# Autodesk Inventor assembly: Drive Roller Assembly 3 (Lexan)
(part 2 of 2)
- Flush:42: Hex Shaft Collar 3-8 in (7552K300):3 ↔ Hex Shaft 3-8 in (am-0855):4
- Mate:1246: Vex Pro 1x1 rectangular tubing 14 in length:5 ↔ Vex Pro T gusset - OUT OF STOCK 1192014:3
- Mate:1247: Vex Pro 1x1 rectangular tubing 14 in length:5 ↔ Vex Pro T gusset - OUT OF STOCK 1192014:3
- Mate:1248: Vex Pro 1x1 rectangular tubing 14 in length:5 ↔ Vex Pro T gusset - OUT OF STOCK 1192014:3
- Mate:1249: Vex Pro 1x1 rectangular tubing 4 in length:1 ↔ Vex Pro T gusset - OUT OF STOCK 1192014:3
- Mate:1250: Vex Pro 1x1 rectangular tubing 14 in length:5 ↔ Vex Pro T gusset - OUT OF STOCK 1192014:4
- Mate:1251: Vex Pro 1x1 rectangular tubing 14 in length:5 ↔ Vex Pro T gusset - OUT OF STOCK 1192014:4
- Mate:1252: Vex Pro 1x1 rectangular tubing 14 in length:5 ↔ Vex Pro T gusset - OUT OF STOCK 1192014:4
- Mate:1253: Vex Pro 1x1 rectangular tubing 4 in length:1 ↔ Vex Pro T gusset - OUT OF STOCK 1192014:4
- Mate:1254: Vex Pro 1x1 rectangular tubing 14 in length:6 ↔ Vex Pro T gusset - OUT OF STOCK 1192014:5
- Mate:1255: Vex Pro 1x1 rectangular tubing 14 in length:6 ↔ Vex Pro T gusset - OUT OF STOCK 1192014:5
- Mate:1256: Vex Pro 1x1 rectangular tubing 14 in length:6 ↔ Vex Pro T gusset - OUT OF STOCK 1192014:5
- Mate:1257: Vex Pro 1x1 rectangular tubing 4 in length:2 ↔ Vex Pro T gusset - OUT OF STOCK 1192014:5
- Mate:1258: Vex Pro 1x1 rectangular tubing 4 in length:1 ↔ Vex Pro T gusset - OUT OF STOCK 1192014:3
- Mate:1259: Vex Pro 1x1 rectangular tubing 4 in length:2 ↔ Vex Pro T gusset - OUT OF STOCK 1192014:5
- Mate:1260: Vex Pro 1x1 rectangular tubing 14 in length:6 ↔ Vex Pro T gusset - OUT OF STOCK 1192014:6
- Mate:1261: Vex Pro 1x1 rectangular tubing 14 in length:6 ↔ Vex Pro T gusset - OUT OF STOCK 1192014:6
- Mate:1262: Vex Pro 1x1 rectangular tubing 14 in length:6 ↔ Vex Pro T gusset - OUT OF STOCK 1192014:6
- Mate:1263: Vex Pro 1x1 rectangular tubing 4 in length:2 ↔ Vex Pro T gusset - OUT OF STOCK 1192014:6
- Mate:1264: Vex Pro 1x1 rectangular tubing 4 in length:2 ↔ Vex Pro T gusset - OUT OF STOCK 1192014:6
- Mate:1265: Vex Pro 1x1 rectangular tubing 4 in length:1 ↔ Vex Pro T gusset - OUT OF STOCK 1192014:3
- Mate:1266: Hex Spacer:3 ↔ Clamp with Piston Assembly (new):1
- Mate:1267: Vex Pro 1x1 rectangular tubing 21.375 in length:1 ↔ Roller Crossbar Gusset (Custom):5
- Mate:1268: Vex Pro 1x1 rectangular tubing 21.375 in length:1 ↔ Roller Crossbar Gusset (Custom):5
- Mate:1269: Vex Pro 1x1 rectangular tubing 21.375 in length:1 ↔ Roller Crossbar Gusset (Custom):5
- Mate:1272: Vex Pro 1x1 rectangular tubing 14 in length:5 ↔ Roller Piston 4 Mount:1
- Mate:1273: Vex Pro 1x1 rectangular tubing 14 in length:5 ↔ Roller Piston 4 Mount:1
- Mate:1274: Vex Pro 1x1 rectangular tubing 14 in length:5 ↔ Roller Piston 4 Mount:1
- Mate:1275: Vex Pro 1x1 rectangular tubing 14 in length:6 ↔ Roller Piston 4 Mount:2
- Mate:1276: Vex Pro 1x1 rectangular tubing 14 in length:6 ↔ Roller Piston 4 Mount:2
- Mate:1277: Vex Pro 1x1 rectangular tubing 14 in length:6 ↔ Roller Piston 4 Mount:2
- Mate:1278: Roller Piston 4 Mount:2 ↔ Roller Piston 4 (.5 and 1 in Stroke, 9-16 in Bore):1
- Mate:1279: Roller Piston 4 Mount:2 ↔ Roller Piston 4 (.5 and 1 in Stroke, 9-16 in Bore):1
- Mate:1280: Roller Piston 4 Mount:1 ↔ Roller Piston 4 (.5 and 1 in Stroke, 9-16 in Bore):2
- Mate:1281: Roller Piston 4 Mount:1 ↔ Roller Piston 4 (.5 and 1 in Stroke, 9-16 in Bore):2
- Mate:1282: Bracket:3 ↔ Roller Piston 4 (.5 and 1 in Stroke, 9-16 in Bore):2
- Mate:1283: Shaft Collar 3-16 in ID (6435K510):2 ↔ Roller Piston 4 (.5 and 1 in Stroke, 9-16 in Bore):2
- Mate:1284: Shaft Collar 3-16 in ID (6435K510):1 ↔ Roller Piston 4 (.5 and 1 in Stroke, 9-16 in Bore):2
- Mate:1285: Bracket:4 ↔ Roller Piston 4 (.5 and 1 in Stroke, 9-16 in Bore):1
- Mate:1286: Shaft Collar 3-16 in ID (6435K510):4 ↔ Roller Piston 4 (.5 and 1 in Stroke, 9-16 in Bore):1
- Mate:1287: Shaft Collar 3-16 in ID (6435K510):3 ↔ Roller Piston 4 (.5 and 1 in Stroke, 9-16 in Bore):1
- Mate:1292: Vex Pro 1x1 rectangular tubing 14 in length:6 ↔ Vex Pro T gusset - OUT OF STOCK 1192014:8
- Mate:1293: Vex Pro 1x1 rectangular tubing 14 in length:6 ↔ Vex Pro T gusset - OUT OF STOCK 1192014:8
- Mate:1294: Vex Pro 1x1 rectangular tubing 14 in length:6 ↔ Vex Pro T gusset - OUT OF STOCK 1192014:8
- Mate:1300: Hex Shaft Collar 1-2 in (7552K500):19 ↔ Hex Shaft 1-2 in 5 in long (am-0856):1
- Mate:1301: Hex Shaft Collar 1-2 in (7552K500):18 ↔ Hex Shaft 1-2 in 5 in long (am-0856):1
- Mate:1306: Pneumatic Piston Front Flange (Rt Custom):2 ↔ Clamp Piston Right Mount:1
- Mate:1307: Pneumatic Piston Front Flange (Rt Custom):2 ↔ Clamp Piston Right Mount:1
- Mate:1308: Pneumatic Piston Front Flange (Rt Custom):2 ↔ Clamp Piston Right Mount:1
- Mate:1309: Clamp with Piston Assembly (new):2 ↔ Vex Pro 90 degree gusset (1-8 in):5
- Mate:1310: Clamp with Piston Assembly (new):2 ↔ Vex Pro 90 degree gusset (1-8 in):5
- Mate:1312: Clamp with Piston Assembly (new):1 ↔ Vex Pro 90 degree gusset (1-8 in):6
- Mate:1320: Vex Pro 90 degree gusset (1-8 in):6 ↔ Vex Pro 1x1 rectangular tubing 2 in length (no hex):3
- Mate:1323: Vex Pro 90 degree gusset (1-8 in):5 ↔ Vex Pro 1x1 rectangular tubing 2 in length (no hex):4
- Mate:1326: Clamp with Piston Assembly (new):2 ↔ Pneumatic Piston Front Flange (Rt Custom):3
- Mate:1327: Clamp with Piston Assembly (new):2 ↔ Pneumatic Piston Front Flange (Rt Custom):3
- Mate:1328: Clamp with Piston Assembly (new):2 ↔ Pneumatic Piston Front Flange (Rt Custom):3
- Mate:1329: Clamp Piston Left Mount:1 ↔ Pneumatic Piston Front Flange (Rt Custom):3
- Mate:1330: Clamp Piston Left Mount:1 ↔ Pneumatic Piston Front Flange (Rt Custom):3
- Mate:1331: Clamp Piston Left Mount:1 ↔ Pneumatic Piston Front Flange (Rt Custom):3
- Mate:1337: Vex Pro T gusset - OUT OF STOCK 1192014:2 ↔ Vex Pro 1x1 rectangular tubing 2 in length (no hex, eyebolt):1
- Flush:44: Vex Pro T gusset - OUT OF STOCK 1192014:2 ↔ Vex Pro 1x1 rectangular tubing 2 in length (no hex, eyebolt):1
- Mate:1338: Steel Eyebolt (3014T102):1 ↔ Vex Pro 1x1 rectangular tubing 2 in length (no hex, eyebolt):1
- Mate:1339: Steel Eyebolt (3014T102):1 ↔ Vex Pro 1x1 rectangular tubing 2 in length (no hex, eyebolt):1
- Mate:1340: Vex Pro T gusset - OUT OF STOCK 1192014:8 ↔ Vex Pro 1x1 rectangular tubing 2 in length (no hex, eyebolt):2
- Mate:1341: Vex Pro T gusset - OUT OF STOCK 1192014:8 ↔ Vex Pro 1x1 rectangular tubing 2 in length (no hex, eyebolt):2
- Flush:45: Vex Pro T gusset - OUT OF STOCK 1192014:8 ↔ Vex Pro 1x1 rectangular tubing 2 in length (no hex, eyebolt):2
- Mate:1342: Vex Pro 1x1 rectangular tubing 2 in length (no hex, eyebolt):2 ↔ Steel Eyebolt (3014T102):2
- Mate:1343: Vex Pro 1x1 rectangular tubing 2 in length (no hex, eyebolt):2 ↔ Steel Eyebolt (3014T102):2
- Mate:1344: Clamp with Piston Assembly (new):1 ↔ Vex Pro 90 degree gusset (1-8 in):6
- Mate:1345: Clamp with Piston Assembly (new):1 ↔ Vex Pro 90 degree gusset (1-8 in):6
- Mate:1346: Vex Pro 90 degree gusset (1-8 in):6 ↔ Vex Pro 1x1 rectangular tubing 2 in length (no hex):3
- Mate:1347: Vex Pro 90 degree gusset (1-8 in):6 ↔ Vex Pro 1x1 rectangular tubing 2 in length (no hex):3
- Mate:1348: Clamp with Piston Assembly (new):2 ↔ Vex Pro 90 degree gusset (1-8 in):5
- Mate:1349: Vex Pro 90 degree gusset (1-8 in):5 ↔ Vex Pro 1x1 rectangular tubing 2 in length (no hex):4
- Mate:1350: Vex Pro 90 degree gusset (1-8 in):5 ↔ Vex Pro 1x1 rectangular tubing 2 in length (no hex):4
- Mate:1351: Vex Pro 1x1 rectangular tubing 4 in length:4 ↔ Steel Eyebolt 3-8 in (3014T142):1
- Mate:1352: Vex Pro 1x1 rectangular tubing 4 in length:4 ↔ Steel Eyebolt 3-8 in (3014T142):1
- Mate:1353: Vex Pro 1x1 rectangular tubing 4 in length:3 ↔ Steel Eyebolt 3-8 in (3014T142):2
- Mate:1354: Vex Pro 1x1 rectangular tubing 4 in length:3 ↔ Steel Eyebolt 3-8 in (3014T142):2
- Mate:1355: Steel Eyebolt 3-8 in (3014T142):2 ↔ Locknut 3-8 in (97135A230):1
- Mate:1356: Vex Pro 1x1 rectangular tubing 4 in length:3 ↔ Locknut 3-8 in (97135A230):1
- Mate:1357: Steel Eyebolt 3-8 in (3014T142):1 ↔ Locknut 3-8 in (97135A230):2
- Mate:1359: Hex Shaft Collar 1-2 in (7552K500):19 ↔ Hex Shaft 1-2 in 5 in long (am-0856):1
- Mate:1360: Hex Shaft Collar 1-2 in (7552K500):19 ↔ Hex Shaft 1-2 in 5 in long (am-0856):1
- Mate:1361: Hex Shaft Collar 1-2 in (7552K500):18 ↔ Hex Shaft 1-2 in 5 in long (am-0856):1
- Mate:1362: Pneumatic Piston Back Flange (Rt Custom):1 ↔ Clamp Piston ( 1 in stroke twice, 9-16 bore):1
- Mate:1363: Pneumatic Piston Back Flange (Rt Custom):1 ↔ Clamp Piston ( 1 in stroke twice, 9-16 bore):1
- Mate:1364: Pneumatic Piston Back Flange (Rt Custom):1 ↔ Clamp Piston ( 1 in stroke twice, 9-16 bore):1
- Mate:1365: Clamp Piston Left Mount:1 ↔ Clamp Piston ( 1 in stroke twice, 9-16 bore):1
- Mate:1366: Pneumatic Piston Back Flange (Right Custom):1 ↔ Clamp Piston ( 1 in stroke twice, 9-16 bore):2
- Mate:1367: Pneumatic Piston Back Flange (Right Custom):1 ↔ Clamp Piston ( 1 in stroke twice, 9-16 bore):2
- Mate:1368: Pneumatic Piston Back Flange (Right Custom):1 ↔ Clamp Piston ( 1 in stroke twice, 9-16 bore):2
- Mate:1369: Roller Piston 4 Mount:2 ↔ Vex Pro 1x1 rectangular tubing 4 in length:4
- Flush:46: Roller Piston 4 Mount:2 ↔ Vex Pro 1x1 rectangular tubing 4 in length:4
- Mate:1370: Roller Piston 4 Mount:2 ↔ Vex Pro 1x1 rectangular tubing 4 in length:4
- Mate:1371: Vex Pro 1x1 rectangular tubing 14 in length:5 ↔ Vex Pro 90 degree gusset (1-8 in):2
- Mate:1372: Lexan flexible Arm Mount:4 ↔ Hex Shaft Connector Pivot:1
- Mate:1373: Lexan flexible Arm Mount:4 ↔ Hex Shaft Connector Pivot:1
- Mate:1374: Lexan flexible Arm Mount:4 ↔ Hex Shaft Connector Pivot:1
- Mate:1375: Lexan flexible Arm Mount:3 ↔ Hex Shaft Connector Pivot:2
- Mate:1376: Lexan flexible Arm Mount:3 ↔ Hex Shaft Connector Pivot:2
- Mate:1377: Lexan flexible Arm Mount:3 ↔ Hex Shaft Connector Pivot:2
- Mate:1378: Lexan flexible Arm Mount:1 ↔ Hex Shaft Connector Pivot:3
- Mate:1379: Lexan flexible Arm Mount:1 ↔ Hex Shaft Connector Pivot:3
- Mate:1380: Lexan flexible Arm Mount:1 ↔ Hex Shaft Connector Pivot:3
- Mate:1381: Lexan flexible Arm Mount:2 ↔ Hex Shaft Connector Pivot:4
- Mate:1382: Lexan flexible Arm Mount:2 ↔ Hex Shaft Connector Pivot:4
- Mate:1383: Lexan flexible Arm Mount:2 ↔ Hex Shaft Connector Pivot:4
- Mate:1384: Hex Shaft Collar 1-2 in (7552K500):30 ↔ Hex Shaft Connector Pivot:4
- Mate:1385: Hex Shaft Collar 1-2 in (7552K500):21 ↔ Hex Shaft Connector Pivot:3
- Mate:1386: Hex Shaft Collar 1-2 in (7552K500):19 ↔ Hex Shaft Connector Pivot:1
- Mate:1387: Hex Shaft Collar 1-2 in (7552K500):18 ↔ Hex Shaft Connector Pivot:2
- Mate:1388: Hex Shaft 1-2 in 5 in long (am-0856):1 ↔ Lexan flexible Arm Mount:3
- Mate:1389: Hex Shaft 1-2 in 5 in long (am-0856):1 ↔ Lexan flexible Arm Mount:3
## Named parameters: d240_d195 = 0 mm, d241_d196 = 0 mm, d242_d197 = 0 mm, d243_d198 = 0 mm, d305_d302 = 0 mm, d306_d303 = 0 mm, d307_d304 = 0 mm, d334_d317 = 0 mm, d339_d304 = 0 mm, d343_d308 = 0 mm, d344_d309 = 0 mm, d345_d310 = 0 mm, d346_d316 = 0 mm, d349_d328 = 0 mm, d350_d329 = 0 mm, d352_d331 = 0 mm, d353_d332 = 0 mm, d770_d743 = 0 mm, d771_d744 = 0 mm, d772_d745 = 0 mm, d773_d746 = 0 mm, d791_d742 = 0 mm, d1331_d1327 = 0 mm, d1332_d1328 = 0 mm
